# Autodesk Inventor assembly: Main Assem
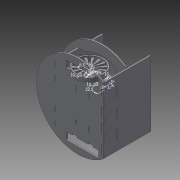
[picture p0: Inventor's stored thumbnail of the model, 180x180]
Saved by Autodesk Inventor 2015 (Build 190159000, 159)
## iProperties
Created: 2014-07-26
Part Number: Main Assem
Document SubType Name: Assembly
Designer: karl
Author: karl
## Documents named in this file (9)
- C:\Users\karl\Documents\GitHub\SUMOChasis\Body\Main frame\Main Assem.iam
- C:\Users\karl\Documents\GitHub\SUMOChasis\Body\Main frame\BasePlate.ipt
- C:\Users\karl\Documents\GitHub\SUMOChasis\Body\Main frame\Motor mount.ipt
- C:\Users\karl\Documents\GitHub\SUMOChasis\Body\Main frame\Wheel.ipt
- C:\Users\karl\Documents\GitHub\SUMOChasis\Body\Main frame\Motor side.ipt
- C:\Users\karl\Documents\GitHub\SUMOChasis\Body\Main frame\frount plate.ipt
- C:\Users\karl\Documents\GitHub\SUMOChasis\Body\Main frame\Mid Plate.ipt
- C:\Users\karl\Documents\GitHub\SUMOChasis\Body\Back support.ipt
- C:\Users\karl\Documents\GitHub\SUMOChasis\Body\suport plate.ipt
## Components (10 placed, 8 different names)
1. BasePlate:1 — Flush:1, Mate:1, Flush:2, Mate:5, Mate:7, Flush:6, Mate:8, Mate:11, Mate:12, Mate:15
2. Motor mount:1 — Flush:1, Mate:1, Flush:2, Mate:2, Mate:3, Mate:4, Flush:3, Flush:4, Mate:6, Flush:7
3. Wheel:1 — Mate:2, Mate:3
4. Motor side:1 — Mate:4, Mate:5, Flush:3, Flush:5, Flush:8
5. Motor side:2 — Flush:4, Flush:5, Mate:6
6. frount plate:1 — Mate:7, Flush:6, Mate:8, Mate:9, Mate:14
7. Power distabution plate — Flush:7, Mate:9, Flush:8, Flush:9, Mate:10, Flush:10, Mate:13, Mate:16
8. Back support:1 — Flush:9, Mate:10, Mate:11
9. Back support:2 — Flush:10, Mate:12, Mate:13
10. suport plate:1 — Mate:14, Mate:15, Mate:16
## Relationships (26: Mate 16, Flush 10)
- Flush:1: BasePlate:1 ↔ Motor mount:1
- Mate:1: BasePlate:1 ↔ Motor mount:1
- Flush:2: BasePlate:1 ↔ Motor mount:1
- Mate:2: Motor mount:1 ↔ Wheel:1
- Mate:3 (3 mm): Motor mount:1 ↔ Wheel:1
- Mate:4: Motor mount:1 ↔ Motor side:1
- Mate:5: BasePlate:1 ↔ Motor side:1
- Flush:3: Motor mount:1 ↔ Motor side:1
- Flush:4: Motor mount:1 ↔ Motor side:2
- Flush:5: Motor side:1 ↔ Motor side:2
- Mate:6: Motor mount:1 ↔ Motor side:2
- Mate:7: BasePlate:1 ↔ frount plate:1
- Flush:6: BasePlate:1 ↔ frount plate:1
- Mate:8: BasePlate:1 ↔ frount plate:1
- Flush:7: Motor mount:1 ↔ Power distabution plate
- Mate:9: frount plate:1 ↔ Power distabution plate
- Flush:8: Motor side:1 ↔ Power distabution plate
- Flush:9: Power distabution plate ↔ Back support:1
- Mate:10: Power distabution plate ↔ Back support:1
- Mate:11: BasePlate:1 ↔ Back support:1
- Flush:10: Power distabution plate ↔ Back support:2
- Mate:12: BasePlate:1 ↔ Back support:2
- Mate:13: Power distabution plate ↔ Back support:2
- Mate:14: frount plate:1 ↔ suport plate:1
- Mate:15: BasePlate:1 ↔ suport plate:1
- Mate:16 (20 mm): Power distabution plate ↔ suport plate:1
